# Autodesk Inventor assembly: Cartridge Assembly 2
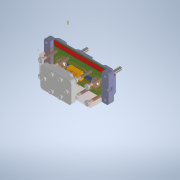
[picture p0: Inventor's stored thumbnail of the model, 180x180]
Saved by Autodesk Inventor 2021 (Build 250183000, 183)
## iProperties
Created: 2020-04-22
Part Number: Cartridge Assembly 2
Document SubType Name: Assembly
Designer: jgray
Author: jgray
## Documents named in this file (12)
- M:\Printed Electronics\Gas Sensors\Prototypes\Prototype II -Cartridge Reader V2\Cartridge Interface V5 30-06-20\Cartridge Assembly 2.iam
- M:\Printed Electronics\Gas Sensors\Prototypes\Prototype II -Cartridge Reader V2\Cartridge Interface V5 30-06-20\Cartridge PCB Assembly.iam
- M:\Printed Electronics\Gas Sensors\Prototypes\Prototype II -Cartridge Reader V2\Cartridge Interface V5 30-06-20\Device Chiplet.ipt
- M:\Printed Electronics\Gas Sensors\Prototypes\Prototype II -Cartridge Reader V2\Cartridge Interface V5 30-06-20\RS 278-534 M3 fixing Dia4FixHole.ipt
- M:\Printed Electronics\Gas Sensors\Prototypes\Prototype II -Cartridge Reader V2\Cartridge Interface V5 30-06-20\DIN 7985 (H) - M3x25-H.ipt
- M:\Printed Electronics\Gas Sensors\Prototypes\Prototype II -Cartridge Reader V2\Cartridge Interface V5 30-06-20\DIN 7985 (H) - M3x16-H.ipt
- M:\Printed Electronics\Gas Sensors\Prototypes\Prototype II -Cartridge Reader V2\Cartridge Interface V5 30-06-20\DIN 6798 - J 3.2.ipt
- M:\Printed Electronics\Gas Sensors\Prototypes\Prototype II -Cartridge Reader V2\Cartridge Interface V5 30-06-20\Cartridge Internal - Top Cover 2.ipt
- M:\Printed Electronics\Gas Sensors\Prototypes\Prototype II -Cartridge Reader V2\Cartridge Interface V5 30-06-20\Top Seal 1.ipt
- M:\Printed Electronics\Gas Sensors\Prototypes\Prototype II -Cartridge Reader V2\Cartridge Interface V5 30-06-20\Base Seal.ipt
- M:\Printed Electronics\Gas Sensors\Prototypes\Prototype II -Cartridge Reader V2\Cartridge Interface V5 30-06-20\Cartridge interface plate 8-7-20-5.ipt
- M:\Printed Electronics\Gas Sensors\Prototypes\Prototype II -Cartridge Reader V2\Cartridge Interface V5 30-06-20\Cartridge Mid-Cover 2 Mach 7-7-20-5.ipt
## Components (50 placed, 11 different names)
1. Cartridge interface plate 8-7-20-5:1 — Angle:1, Angle:2, Mate:1, Mate:2, Mate:3, Mate:19, Flush:14, Flush:15, Flush:16, Flush:17, Flush:18, Flush:19, Flush:20, Flush:21
2. Cartridge PCB Assembly:1 [sub-assembly] — Mate:1, Mate:2, Mate:3, Mate:4, Flush:6, Mate:5, Mate:6, Flush:7, Mate:7, Mate:9, Mate:10
3. Device Chiplet:1 — Mate:6, Flush:7, Mate:7
4. Device Chiplet:2 — Mate:4, Flush:6, Mate:5
5. Cartridge Mid-Cover 2 Mach 7-7-20-5:1 — Mate:9, Mate:10, Mate:11, Mate:12, Mate:13, Mate:14, Mate:15, Mate:16, Flush:8, Flush:9, Flush:10, Flush:11, Flush:12, Flush:13, Mate:19, Mate:21, Mate:22, Mate:23, Mate:24, Mate:25, Mate:26, Mate:27, Mate:28, Mate:29, Mate:30, Mate:31, Mate:32, Mate:33, Mate:34, Mate:35, Mate:36, Mate:45, Mate:46, Mate:47, Mate:48, Mate:49, Mate:50, Mate:51, Mate:86, Mate:87, Mate:88, Mate:113, Mate:114, Mate:115, Mate:116, Mate:117, Mate:118
6. RS 278-534 M3 fixing Dia4FixHole:1 — Mate:11, Flush:8
7. RS 278-534 M3 fixing Dia4FixHole:2 — Mate:12, Flush:13
8. RS 278-534 M3 fixing Dia4FixHole:3 — Mate:13, Flush:12
9. RS 278-534 M3 fixing Dia4FixHole:4 — Mate:14, Flush:11
10. RS 278-534 M3 fixing Dia4FixHole:5 — Mate:15, Flush:10
11. RS 278-534 M3 fixing Dia4FixHole:6 — Mate:16, Flush:9
12. DIN 7985 (H) M3x25-H:1 — Mate:38, Mate:51, Mate:78
13. DIN 7985 (H) M3x25-H:2 — Mate:37, Mate:52, Mate:77
14. DIN 7985 (H) M3x25-H:3 — Mate:39, Mate:49, Mate:80
15. DIN 7985 (H) M3x25-H:4 — Mate:40, Mate:50, Mate:79
16. DIN 7985 (H) M3x25-H:5 — Mate:41, Mate:48, Mate:82
17. DIN 7985 (H) M3x25-H:6 — Mate:42, Mate:47, Mate:81
18. DIN 7985 (H) M3x25-H:8 — Mate:44, Mate:45, Mate:83
19. DIN 7985 (H) M3x25-H:9 — Mate:43, Mate:46, Mate:84
20. DIN 7985 (H) M3x16-H:1 — Mate:91, Mate:100, Mate:107
21. DIN 7985 (H) M3x16-H:2 — Mate:90, Mate:99, Mate:109
22. DIN 7985 (H) M3x16-H:3 — Mate:92, Mate:98, Mate:108
23. DIN 7985 (H) M3x16-H:4 — Mate:89, Mate:97, Mate:110
24. DIN 7985 (H) M3x16-H:5 — Mate:93, Mate:96, Mate:112
25. DIN 7985 (H) M3x16-H:6 — Mate:94, Mate:95, Mate:111
26. DIN 6798 J J 3.2:2 — Mate:22, Mate:27, Mate:43
27. DIN 6798 J J 3.2:3 — Mate:33, Mate:36, Mate:37, Mate:52
28. DIN 6798 J J 3.2:4 — Mate:23, Mate:30, Mate:39
29. DIN 6798 J J 3.2:5 — Mate:21, Mate:28, Mate:42
30. DIN 6798 J J 3.2:6 — Mate:32, Mate:35, Mate:38
31. DIN 6798 J J 3.2:7 — Mate:91, Mate:106, Mate:107
32. DIN 6798 J J 3.2:8 — Mate:31, Mate:34, Mate:40
33. DIN 6798 J J 3.2:9 — Mate:25, Mate:29, Mate:41
34. DIN 6798 J J 3.2:10 — Mate:90, Mate:103, Mate:109
35. DIN 6798 J J 3.2:11 — Mate:94, Mate:102, Mate:111
36. DIN 6798 J J 3.2:12 — Mate:93, Mate:105, Mate:112
37. DIN 6798 J J 3.2:13 — Mate:24, Mate:26, Mate:44
38. DIN 6798 J J 3.2:14 — Mate:92, Mate:104, Mate:108
39. DIN 6798 J J 3.2:15 — Mate:89, Mate:101, Mate:110
40. RS 278-534 M3 fixing Dia4FixHole:7 — Mate:84, Flush:14
41. RS 278-534 M3 fixing Dia4FixHole:8 — Mate:80, Flush:19
42. RS 278-534 M3 fixing Dia4FixHole:9 — Mate:81, Flush:17
43. RS 278-534 M3 fixing Dia4FixHole:10 — Mate:83, Flush:15
44. RS 278-534 M3 fixing Dia4FixHole:11 — Mate:82, Flush:16
45. RS 278-534 M3 fixing Dia4FixHole:12 — Mate:79, Flush:20
46. RS 278-534 M3 fixing Dia4FixHole:13 — Mate:77, Flush:18
47. RS 278-534 M3 fixing Dia4FixHole:14 — Mate:78, Flush:21
48. Cartridge Internal - Top Cover 2:1 — Mate:86, Mate:87, Mate:88, Mate:95, Mate:96, Mate:97, Mate:98, Mate:99, Mate:100, Mate:101, Mate:102, Mate:103, Mate:104, Mate:105, Mate:106
49. Top Seal 1:1 — Mate:113, Mate:114, Mate:115
50. Base Seal:1 — Mate:116, Mate:117, Mate:118
## Relationships (107: Mate 89, Flush 16, Angle 2)
- Angle:1 (0 deg): Cartridge interface plate 8-7-20-5:1
- Angle:2 (180 deg): Cartridge interface plate 8-7-20-5:1
- Mate:1: Cartridge interface plate 8-7-20-5:1 ↔ Cartridge PCB Assembly:1
- Mate:2: Cartridge interface plate 8-7-20-5:1 ↔ Cartridge PCB Assembly:1
- Mate:3: Cartridge interface plate 8-7-20-5:1 ↔ Cartridge PCB Assembly:1
- Mate:4: Cartridge PCB Assembly:1 ↔ Device Chiplet:2
- Flush:6: Cartridge PCB Assembly:1 ↔ Device Chiplet:2
- Mate:5: Cartridge PCB Assembly:1 ↔ Device Chiplet:2
- Mate:6: Cartridge PCB Assembly:1 ↔ Device Chiplet:1
- Flush:7: Cartridge PCB Assembly:1 ↔ Device Chiplet:1
- Mate:7: Cartridge PCB Assembly:1 ↔ Device Chiplet:1
- Mate:9: Cartridge PCB Assembly:1 ↔ Cartridge Mid-Cover 2 Mach 7-7-20-5:1
- Mate:10: Cartridge PCB Assembly:1 ↔ Cartridge Mid-Cover 2 Mach 7-7-20-5:1
- Mate:11: Cartridge Mid-Cover 2 Mach 7-7-20-5:1 ↔ RS 278-534 M3 fixing Dia4FixHole:1
- Mate:12: Cartridge Mid-Cover 2 Mach 7-7-20-5:1 ↔ RS 278-534 M3 fixing Dia4FixHole:2
- Mate:13: Cartridge Mid-Cover 2 Mach 7-7-20-5:1 ↔ RS 278-534 M3 fixing Dia4FixHole:3
- Mate:14: Cartridge Mid-Cover 2 Mach 7-7-20-5:1 ↔ RS 278-534 M3 fixing Dia4FixHole:4
- Mate:15: Cartridge Mid-Cover 2 Mach 7-7-20-5:1 ↔ RS 278-534 M3 fixing Dia4FixHole:5
- Mate:16: Cartridge Mid-Cover 2 Mach 7-7-20-5:1 ↔ RS 278-534 M3 fixing Dia4FixHole:6
- Flush:8 (0.5 mm): Cartridge Mid-Cover 2 Mach 7-7-20-5:1 ↔ RS 278-534 M3 fixing Dia4FixHole:1
- Flush:9 (0.5 mm): Cartridge Mid-Cover 2 Mach 7-7-20-5:1 ↔ RS 278-534 M3 fixing Dia4FixHole:6
- Flush:10 (0.5 mm): Cartridge Mid-Cover 2 Mach 7-7-20-5:1 ↔ RS 278-534 M3 fixing Dia4FixHole:5
- Flush:11 (0.5 mm): Cartridge Mid-Cover 2 Mach 7-7-20-5:1 ↔ RS 278-534 M3 fixing Dia4FixHole:4
- Flush:12 (0.5 mm): Cartridge Mid-Cover 2 Mach 7-7-20-5:1 ↔ RS 278-534 M3 fixing Dia4FixHole:3
- Flush:13 (0.5 mm): Cartridge Mid-Cover 2 Mach 7-7-20-5:1 ↔ RS 278-534 M3 fixing Dia4FixHole:2
- Mate:19: Cartridge interface plate 8-7-20-5:1 ↔ Cartridge Mid-Cover 2 Mach 7-7-20-5:1
- Mate:21: Cartridge Mid-Cover 2 Mach 7-7-20-5:1 ↔ DIN 6798 J J 3.2:5
- Mate:22: Cartridge Mid-Cover 2 Mach 7-7-20-5:1 ↔ DIN 6798 J J 3.2:2
- Mate:23: Cartridge Mid-Cover 2 Mach 7-7-20-5:1 ↔ DIN 6798 J J 3.2:4
- Mate:24: Cartridge Mid-Cover 2 Mach 7-7-20-5:1 ↔ DIN 6798 J J 3.2:13
- Mate:25: Cartridge Mid-Cover 2 Mach 7-7-20-5:1 ↔ DIN 6798 J J 3.2:9
- Mate:26: Cartridge Mid-Cover 2 Mach 7-7-20-5:1 ↔ DIN 6798 J J 3.2:13
- Mate:27: Cartridge Mid-Cover 2 Mach 7-7-20-5:1 ↔ DIN 6798 J J 3.2:2
- Mate:28: Cartridge Mid-Cover 2 Mach 7-7-20-5:1 ↔ DIN 6798 J J 3.2:5
- Mate:29: Cartridge Mid-Cover 2 Mach 7-7-20-5:1 ↔ DIN 6798 J J 3.2:9
- Mate:30: Cartridge Mid-Cover 2 Mach 7-7-20-5:1 ↔ DIN 6798 J J 3.2:4
- Mate:31: Cartridge Mid-Cover 2 Mach 7-7-20-5:1 ↔ DIN 6798 J J 3.2:8
- Mate:32: Cartridge Mid-Cover 2 Mach 7-7-20-5:1 ↔ DIN 6798 J J 3.2:6
- Mate:33: Cartridge Mid-Cover 2 Mach 7-7-20-5:1 ↔ DIN 6798 J J 3.2:3
- Mate:34: Cartridge Mid-Cover 2 Mach 7-7-20-5:1 ↔ DIN 6798 J J 3.2:8
- Mate:35: Cartridge Mid-Cover 2 Mach 7-7-20-5:1 ↔ DIN 6798 J J 3.2:6
- Mate:36: Cartridge Mid-Cover 2 Mach 7-7-20-5:1 ↔ DIN 6798 J J 3.2:3
- Mate:37: DIN 7985 (H) M3x25-H:2 ↔ DIN 6798 J J 3.2:3
- Mate:38: DIN 7985 (H) M3x25-H:1 ↔ DIN 6798 J J 3.2:6
- Mate:39: DIN 7985 (H) M3x25-H:3 ↔ DIN 6798 J J 3.2:4
- Mate:40: DIN 7985 (H) M3x25-H:4 ↔ DIN 6798 J J 3.2:8
- Mate:41: DIN 7985 (H) M3x25-H:5 ↔ DIN 6798 J J 3.2:9
- Mate:42: DIN 7985 (H) M3x25-H:6 ↔ DIN 6798 J J 3.2:5
- Mate:43: DIN 7985 (H) M3x25-H:9 ↔ DIN 6798 J J 3.2:2
- Mate:44: DIN 7985 (H) M3x25-H:8 ↔ DIN 6798 J J 3.2:13
- Mate:45: Cartridge Mid-Cover 2 Mach 7-7-20-5:1 ↔ DIN 7985 (H) M3x25-H:8
- Mate:46: Cartridge Mid-Cover 2 Mach 7-7-20-5:1 ↔ DIN 7985 (H) M3x25-H:9
- Mate:47: Cartridge Mid-Cover 2 Mach 7-7-20-5:1 ↔ DIN 7985 (H) M3x25-H:6
- Mate:48: Cartridge Mid-Cover 2 Mach 7-7-20-5:1 ↔ DIN 7985 (H) M3x25-H:5
- Mate:49: Cartridge Mid-Cover 2 Mach 7-7-20-5:1 ↔ DIN 7985 (H) M3x25-H:3
- Mate:50: Cartridge Mid-Cover 2 Mach 7-7-20-5:1 ↔ DIN 7985 (H) M3x25-H:4
- Mate:51: Cartridge Mid-Cover 2 Mach 7-7-20-5:1 ↔ DIN 7985 (H) M3x25-H:1
- Mate:52: DIN 7985 (H) M3x25-H:2 ↔ DIN 6798 J J 3.2:3
- Mate:77: DIN 7985 (H) M3x25-H:2 ↔ RS 278-534 M3 fixing Dia4FixHole:13
- Mate:78: DIN 7985 (H) M3x25-H:1 ↔ RS 278-534 M3 fixing Dia4FixHole:14
- Mate:79: DIN 7985 (H) M3x25-H:4 ↔ RS 278-534 M3 fixing Dia4FixHole:12
- Mate:80: DIN 7985 (H) M3x25-H:3 ↔ RS 278-534 M3 fixing Dia4FixHole:8
- Mate:81: DIN 7985 (H) M3x25-H:6 ↔ RS 278-534 M3 fixing Dia4FixHole:9
- Mate:82: DIN 7985 (H) M3x25-H:5 ↔ RS 278-534 M3 fixing Dia4FixHole:11
- Mate:83: DIN 7985 (H) M3x25-H:8 ↔ RS 278-534 M3 fixing Dia4FixHole:10
- Mate:84: DIN 7985 (H) M3x25-H:9 ↔ RS 278-534 M3 fixing Dia4FixHole:7
- Flush:14: Cartridge interface plate 8-7-20-5:1 ↔ RS 278-534 M3 fixing Dia4FixHole:7
- Flush:15: Cartridge interface plate 8-7-20-5:1 ↔ RS 278-534 M3 fixing Dia4FixHole:10
- Flush:16: Cartridge interface plate 8-7-20-5:1 ↔ RS 278-534 M3 fixing Dia4FixHole:11
- Flush:17: Cartridge interface plate 8-7-20-5:1 ↔ RS 278-534 M3 fixing Dia4FixHole:9
- Flush:18: Cartridge interface plate 8-7-20-5:1 ↔ RS 278-534 M3 fixing Dia4FixHole:13
- Flush:19: Cartridge interface plate 8-7-20-5:1 ↔ RS 278-534 M3 fixing Dia4FixHole:8
- Flush:20: Cartridge interface plate 8-7-20-5:1 ↔ RS 278-534 M3 fixing Dia4FixHole:12
- Flush:21: Cartridge interface plate 8-7-20-5:1 ↔ RS 278-534 M3 fixing Dia4FixHole:14
- Mate:86: Cartridge Mid-Cover 2 Mach 7-7-20-5:1 ↔ Cartridge Internal - Top Cover 2:1
- Mate:87: Cartridge Mid-Cover 2 Mach 7-7-20-5:1 ↔ Cartridge Internal - Top Cover 2:1
- Mate:88: Cartridge Mid-Cover 2 Mach 7-7-20-5:1 ↔ Cartridge Internal - Top Cover 2:1
- Mate:89: DIN 7985 (H) M3x16-H:4 ↔ DIN 6798 J J 3.2:15
- Mate:90: DIN 7985 (H) M3x16-H:2 ↔ DIN 6798 J J 3.2:10
- Mate:91: DIN 7985 (H) M3x16-H:1 ↔ DIN 6798 J J 3.2:7
- Mate:92: DIN 7985 (H) M3x16-H:3 ↔ DIN 6798 J J 3.2:14
- Mate:93: DIN 7985 (H) M3x16-H:5 ↔ DIN 6798 J J 3.2:12
- Mate:94: DIN 7985 (H) M3x16-H:6 ↔ DIN 6798 J J 3.2:11
- Mate:95: DIN 7985 (H) M3x16-H:6 ↔ Cartridge Internal - Top Cover 2:1
- Mate:96: DIN 7985 (H) M3x16-H:5 ↔ Cartridge Internal - Top Cover 2:1
- Mate:97: DIN 7985 (H) M3x16-H:4 ↔ Cartridge Internal - Top Cover 2:1
- Mate:98: DIN 7985 (H) M3x16-H:3 ↔ Cartridge Internal - Top Cover 2:1
- Mate:99: DIN 7985 (H) M3x16-H:2 ↔ Cartridge Internal - Top Cover 2:1
- Mate:100: DIN 7985 (H) M3x16-H:1 ↔ Cartridge Internal - Top Cover 2:1
- Mate:101: DIN 6798 J J 3.2:15 ↔ Cartridge Internal - Top Cover 2:1
- Mate:102: DIN 6798 J J 3.2:11 ↔ Cartridge Internal - Top Cover 2:1
- Mate:103: DIN 6798 J J 3.2:10 ↔ Cartridge Internal - Top Cover 2:1
- Mate:104: DIN 6798 J J 3.2:14 ↔ Cartridge Internal - Top Cover 2:1
- Mate:105: DIN 6798 J J 3.2:12 ↔ Cartridge Internal - Top Cover 2:1
- Mate:106: DIN 6798 J J 3.2:7 ↔ Cartridge Internal - Top Cover 2:1
- Mate:107: DIN 7985 (H) M3x16-H:1 ↔ DIN 6798 J J 3.2:7
- Mate:108: DIN 7985 (H) M3x16-H:3 ↔ DIN 6798 J J 3.2:14
- Mate:109: DIN 7985 (H) M3x16-H:2 ↔ DIN 6798 J J 3.2:10
- Mate:110: DIN 7985 (H) M3x16-H:4 ↔ DIN 6798 J J 3.2:15
- Mate:111: DIN 7985 (H) M3x16-H:6 ↔ DIN 6798 J J 3.2:11
- Mate:112: DIN 7985 (H) M3x16-H:5 ↔ DIN 6798 J J 3.2:12
- Mate:113 (0.4 mm): Cartridge Mid-Cover 2 Mach 7-7-20-5:1 ↔ Top Seal 1:1
- Mate:114 (0.4 mm): Cartridge Mid-Cover 2 Mach 7-7-20-5:1 ↔ Top Seal 1:1
- Mate:115: Cartridge Mid-Cover 2 Mach 7-7-20-5:1 ↔ Top Seal 1:1
- Mate:116: Cartridge Mid-Cover 2 Mach 7-7-20-5:1 ↔ Base Seal:1
- Mate:117: Cartridge Mid-Cover 2 Mach 7-7-20-5:1 ↔ Base Seal:1
- Mate:118: Cartridge Mid-Cover 2 Mach 7-7-20-5:1 ↔ Base Seal:1
